# Autodesk Inventor assembly: assembly_linear_stepper
Saved by Autodesk Inventor 2021 (Build 250183000, 183)
## iProperties
Created: 2020-12-28
Part Number: assembly_linear_stepper
Document SubType Name: Assembly
Designer: Tomasz
Author: Tomasz
## Documents named in this file (12)
- D:\SynologyDrive\tcodev\tco-cad\mount_camera\mount_camera.iam
- D:\SynologyDrive\tcodev\tco-cad\mount_camera\mount_camera_linear_stepper_base.ipt
- D:\SynologyDrive\tcodev\tco-cad\mount_camera\mount_camera_linear_stepper_carriage.ipt
- D:\SynologyDrive\tcodev\tco-cad\mount_camera\mount_camera_mount_linear_stepper.ipt
- D:\SynologyDrive\tcodev\tco-cad\mount_camera\mount_camera_carriage_top.ipt
- D:\SynologyDrive\tcodev\tco-cad\mount_camera\mount_camera_carriage_bottom.ipt
- D:\SynologyDrive\tcodev\tco-cad\mount_camera\mount_camera_arm_a.ipt
- D:\SynologyDrive\tcodev\tco-cad\mount_camera\mount_camera_arm_b.ipt
- D:\SynologyDrive\tcodev\tco-cad\common\rod.ipt
- D:\SynologyDrive\tcodev\tco-cad\mount_camera\mount_camera_mount_linear_stepper_washer_b.ipt
- D:\SynologyDrive\tcodev\tco-cad\mount_camera\mount_camera_mount_linear_stepper_washer_a.ipt
- D:\SynologyDrive\tcodev\tco-cad\mount_camera\mount_camera_mount_linear_stepper_washer_c.ipt
## Components (11 placed, 11 different names)
1. mount_camera_linear_stepper_base:1 — Mate:1, Flush:1, Mate:2, Mate:3, Mate:4, Mate:22, Mate:23, Mate:24, Mate:25
2. mount_camera_linear_stepper_carriage:1 — Mate:1, Flush:1, Rigid:1, Flush:2
3. mount_camera_mount_linear_stepper:1 — Mate:2, Mate:3, Mate:4, Mate:14, Mate:17, Mate:19, Mate:21
4. mount_camera_carriage_top:1 — Rigid:1, Mate:15, Mate:18
5. mount_camera_carriage_bottom:1 — Flush:2
6. rod:1 — Mate:14
7. mount_camera_arm_a:1 — Mate:15, Mate:18, Mate:20
8. mount_camera_arm_b:1 — Mate:17, Mate:19, Mate:20
9. mount_camera_mount_linear_stepper_washer_b:1 — Mate:24
10. mount_camera_mount_linear_stepper_washer_a:1 — Mate:21, Mate:22, Mate:23
11. mount_camera_mount_linear_stepper_washer_c:1 — Mate:25
## Relationships (18: Mate 15, Flush 2, WeldJoint 1)
- Mate:1: mount_camera_linear_stepper_base:1 ↔ mount_camera_linear_stepper_carriage:1
- Flush:1: mount_camera_linear_stepper_base:1 ↔ mount_camera_linear_stepper_carriage:1
- Mate:2: mount_camera_linear_stepper_base:1 ↔ mount_camera_mount_linear_stepper:1
- Mate:3: mount_camera_linear_stepper_base:1 ↔ mount_camera_mount_linear_stepper:1
- Mate:4: mount_camera_linear_stepper_base:1 ↔ mount_camera_mount_linear_stepper:1
- Rigid:1 [WeldJoint]: mount_camera_linear_stepper_carriage:1 ↔ mount_camera_carriage_top:1
- Flush:2: mount_camera_linear_stepper_carriage:1 ↔ mount_camera_carriage_bottom:1
- Mate:14: mount_camera_mount_linear_stepper:1 ↔ rod:1
- Mate:15: mount_camera_carriage_top:1 ↔ mount_camera_arm_a:1
- Mate:17: mount_camera_mount_linear_stepper:1 ↔ mount_camera_arm_b:1
- Mate:18: mount_camera_carriage_top:1 ↔ mount_camera_arm_a:1
- Mate:19: mount_camera_mount_linear_stepper:1 ↔ mount_camera_arm_b:1
- Mate:20: mount_camera_arm_a:1 ↔ mount_camera_arm_b:1
- Mate:21: mount_camera_mount_linear_stepper:1 ↔ mount_camera_mount_linear_stepper_washer_a:1
- Mate:22: mount_camera_linear_stepper_base:1 ↔ mount_camera_mount_linear_stepper_washer_a:1
- Mate:23: mount_camera_linear_stepper_base:1 ↔ mount_camera_mount_linear_stepper_washer_a:1
- Mate:24: mount_camera_linear_stepper_base:1 ↔ mount_camera_mount_linear_stepper_washer_b:1
- Mate:25: mount_camera_linear_stepper_base:1 ↔ mount_camera_mount_linear_stepper_washer_c:1
